# Autodesk Inventor assembly: 217-2625-100
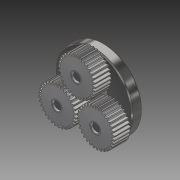
[picture p0: Inventor's stored thumbnail of the model, 180x180]
Saved by Autodesk Inventor 2014 SP1 (Build 180222100, 222)
## iProperties
Created: 2014-01-06
Part Number: 217-2625-100
Document SubType Name: Assembly
Designer: Arpan
Mass: 8.16039 g
Surface Area: 65.7486 cm^2
Volume: 8.16039 cm^3
Density: 1 g/cm^3
Author: Arpan
## Documents named in this file (4)
- C:\Users\Moses\Documents\GitHub\2014buildCAD\Imported Components\217-2 Stage Versaplanetary STEP\217-2625-100.iam
- C:\Users\Moses\Documents\GitHub\2014buildCAD\Imported Components\217-2 Stage Versaplanetary STEP\217-2625-008 Rev1.ipt
- C:\Users\Moses\Documents\GitHub\2014buildCAD\Imported Components\217-2 Stage Versaplanetary STEP\217-2625-010 Rev1.ipt
- C:\Users\Moses\Documents\GitHub\2014buildCAD\Imported Components\217-2 Stage Versaplanetary STEP\217-2625-005 Rev1_Planet_Revolving_Follower01.ipt
## Components (7 placed, 7 different names)
1. 217-2625-008 Rev1_30 — Insert:1, Insert:2, Insert:3
2. 217-2625-010 Rev1_31
3. 217-2625-010 Rev1_32
4. 217-2625-010 Rev1_33
5. 217-2625-005 Rev1_Planet_Revolving_Follower01_34 — Insert:2
6. 217-2625-005 Rev1_Planet_Revolving_Follower01_35 — Insert:3
7. 217-2625-005 Rev1_Planet_Revolving_Follower01_36 — Insert:1
## Relationships (3: Insert 3)
- Insert:1: 217-2625-008 Rev1_30 ↔ 217-2625-005 Rev1_Planet_Revolving_Follower01_36
- Insert:2: 217-2625-008 Rev1_30 ↔ 217-2625-005 Rev1_Planet_Revolving_Follower01_34
- Insert:3: 217-2625-008 Rev1_30 ↔ 217-2625-005 Rev1_Planet_Revolving_Follower01_35
